# Autodesk Inventor assembly: ArmProtoAssembly
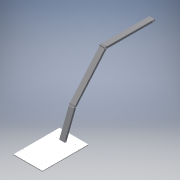
[picture p0: Inventor's stored thumbnail of the model, 180x180]
Saved by Autodesk Inventor 2017 (Build 210142000, 142)
## iProperties
Created: 2017-09-30
Part Number: ArmProtoAssembly
Document SubType Name: Assembly
Designer: User
Author: User
## Documents named in this file (4)
- C:\Robotics\CAD\2017-18_CAD\Miscellaneous\ArmProtoAssembly.iam
- C:\Robotics\CAD\2017-18_CAD\Miscellaneous\ArmProto2.ipt
- C:\Robotics\CAD\2017-18_CAD\PlateFrame1.ipt
- C:\Robotics\CAD\2017-18_CAD\Miscellaneous\ArmProto1.ipt
## Components (4 placed, 3 different names)
1. ArmProto2:1 — Insert:2, Flush:1, Mate:8, Mate:9
2. ArmProto2:2 — Insert:2
3. PlateFrame1:1 — Mate:1, Mate:3, Mate:4, Flush:2, Mate:9
4. ArmProto1:1 — Mate:3, Mate:4, Flush:1, Flush:2, Mate:8
## Relationships (8: Mate 5, Flush 2, Insert 1)
- Insert:2: ArmProto2:1 ↔ ArmProto2:2
- Mate:1: PlateFrame1:1
- Mate:3 (25.4 mm): PlateFrame1:1 ↔ ArmProto1:1
- Mate:4 (-104.14 mm): PlateFrame1:1 ↔ ArmProto1:1
- Flush:1: ArmProto2:1 ↔ ArmProto1:1
- Flush:2 (114.3 mm): PlateFrame1:1 ↔ ArmProto1:1
- Mate:8: ArmProto2:1 ↔ ArmProto1:1
- Mate:9 (-12.7 mm): ArmProto2:1 ↔ PlateFrame1:1
